# Autodesk Inventor assembly: Pancake_Timing Assy_Star Shaft 2_3 Lanes
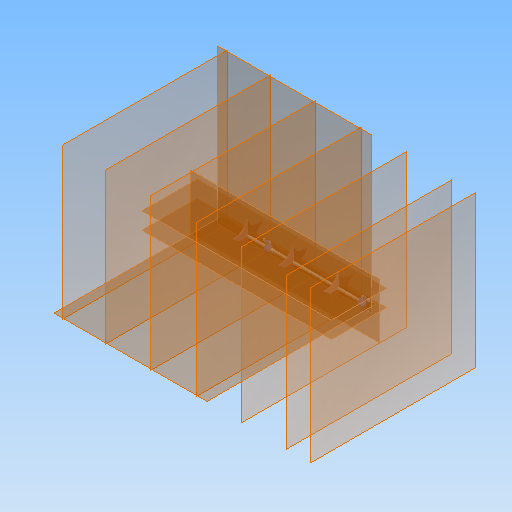
[picture p0: Inventor's stored thumbnail of the model, 512x512]
Saved by Autodesk Inventor 2018.1 (Build 221171000, 171)
## iProperties
Created: 2019-02-11
Part Number: Pancake_Timing Assy_Star Shaft 2_3 Lanes
Document SubType Name: Assembly
Designer: James
Mass: 92.827 g
Surface Area: 261.339 cm^2
Volume: 33.0472 cm^3
Density: 2.80892 g/cm^3
Author: James
## Documents named in this file (7)
- C:\Users\admin\Desktop\Ball-Machine\Pancake Sort\Pancake - 3 Lanes\Pancake_Timing Assy_Star Shaft 2_3 Lanes.iam
- C:\Users\admin\Desktop\Ball-Machine\Pancake Sort\BS 3673 - 6mm External Circlip.ipt
- C:\Users\admin\Desktop\Ball-Machine\Timing Gate\SAFL212 Oval 2 Bolt Flanged Unit.ipt
- C:\Users\admin\Desktop\Ball-Machine\Pancake Sort\Locknut - M3.ipt
- C:\Users\admin\Desktop\Ball-Machine\Pancake Sort\Socket Cap Screw - Standard - (A2) - M3 x 12.ipt
- C:\Users\admin\Desktop\Ball-Machine\Timing Gate\Timing_Star.ipt
- C:\Users\admin\Desktop\Ball-Machine\Pancake Sort\Pancake - 3 Lanes\Pancake_Star Shaft 2_3 Lanes.ipt
## Components (19 placed, 6 different names)
1. Pancake_Star Shaft 2_3 Lanes:1 — Mate:4, Mate:49, Mate:50, Mate:61, Mate:62, Mate:63, Mate:66, Mate:68, Flush:29
2. SAFL212 Oval 2 Bolt Flanged Unit:1 — Mate:61, Flush:24, Angle:4, Mate:65, Mate:79, Mate:80, Mate:81, Mate:82, Mate:83
3. SAFL212 Oval 2 Bolt Flanged Unit:2 — Mate:62, Flush:24, Mate:64, Mate:74, Mate:75, Mate:76, Mate:77, Mate:78, Flush:29
4. BS 3673 - 6mm External Circlip:16 — Mate:65, Mate:66, Flush:25, Mate:68
5. BS 3673 - 6mm External Circlip:17 — Mate:63, Mate:64, Flush:25, Flush:26
6. Locknut - M3:1 — Flush:27, Mate:78
7. Socket Cap Screw - Standard - (A2) - M3 x 12:1 — Mate:74, Mate:77
8. Locknut - M3:2 — Flush:27
9. Socket Cap Screw - Standard - (A2) - M3 x 12:2 — Mate:75, Mate:76
10. Locknut - M3:3 — Flush:28, Mate:83
11. Socket Cap Screw - Standard - (A2) - M3 x 12:3 — Mate:79, Mate:81
12. Locknut - M3:4 — Flush:28
13. Socket Cap Screw - Standard - (A2) - M3 x 12:4 — Mate:80, Mate:82
14. BS 3673 - 6mm External Circlip:11 — Mate:49, Mate:50, Flush:26, Mate:69
15. Timing_Star:1 — Mate:4, Mate:69
16. BS 3673 - 6mm External Circlip:12
17. Timing_Star:2
18. BS 3673 - 6mm External Circlip:13
19. Timing_Star:3
## Component patterns: (3 elements, first: BS 3673 - 6mm External Circlip:11 + Timing_Star:1)
## Relationships (39: Mate 25, Flush 12, Angle 2)
- Mate:4: Pancake_Star Shaft 2_3 Lanes:1 ↔ Timing_Star:1
- [Flush]: Pancake_Star Shaft 2_3 Lanes:1
- Flush:11 (-58 mm)
- Flush:12 (-5 mm)
- Flush:13 (30 mm)
- [Flush]: Pancake_Star Shaft 2_3 Lanes:1
- [Flush]: Pancake_Star Shaft 2_3 Lanes:1
- Mate:49: Pancake_Star Shaft 2_3 Lanes:1 ↔ BS 3673 - 6mm External Circlip:11
- Mate:50: Pancake_Star Shaft 2_3 Lanes:1 ↔ BS 3673 - 6mm External Circlip:11
- [Angle] (0 deg): Pancake_Star Shaft 2_3 Lanes:1 ↔ BS 3673 - 6mm External Circlip:11
- Mate:61: Pancake_Star Shaft 2_3 Lanes:1 ↔ SAFL212 Oval 2 Bolt Flanged Unit:1
- Mate:62: Pancake_Star Shaft 2_3 Lanes:1 ↔ SAFL212 Oval 2 Bolt Flanged Unit:2
- Flush:24: SAFL212 Oval 2 Bolt Flanged Unit:1 ↔ SAFL212 Oval 2 Bolt Flanged Unit:2
- Angle:4 (0 deg): SAFL212 Oval 2 Bolt Flanged Unit:1
- Mate:63: Pancake_Star Shaft 2_3 Lanes:1 ↔ BS 3673 - 6mm External Circlip:17
- Mate:64: SAFL212 Oval 2 Bolt Flanged Unit:2 ↔ BS 3673 - 6mm External Circlip:17
- Mate:65: SAFL212 Oval 2 Bolt Flanged Unit:1 ↔ BS 3673 - 6mm External Circlip:16
- Mate:66: Pancake_Star Shaft 2_3 Lanes:1 ↔ BS 3673 - 6mm External Circlip:16
- Flush:25: BS 3673 - 6mm External Circlip:16 ↔ BS 3673 - 6mm External Circlip:17
- Flush:26: BS 3673 - 6mm External Circlip:17 ↔ BS 3673 - 6mm External Circlip:11
- Mate:69: BS 3673 - 6mm External Circlip:11 ↔ Timing_Star:1
- Mate:68: Pancake_Star Shaft 2_3 Lanes:1 ↔ BS 3673 - 6mm External Circlip:16
- [Mate]: Locknut - M3:1 ↔ Socket Cap Screw - Standard - (A2) - M3 x 12:1
- [Mate]: Locknut - M3:2 ↔ Socket Cap Screw - Standard - (A2) - M3 x 12:2
- [Mate]: Locknut - M3:3 ↔ Socket Cap Screw - Standard - (A2) - M3 x 12:3
- [Mate]: Locknut - M3:4 ↔ Socket Cap Screw - Standard - (A2) - M3 x 12:4
- Mate:74: SAFL212 Oval 2 Bolt Flanged Unit:2 ↔ Socket Cap Screw - Standard - (A2) - M3 x 12:1
- Mate:75: SAFL212 Oval 2 Bolt Flanged Unit:2 ↔ Socket Cap Screw - Standard - (A2) - M3 x 12:2
- Mate:76: SAFL212 Oval 2 Bolt Flanged Unit:2 ↔ Socket Cap Screw - Standard - (A2) - M3 x 12:2
- Mate:77: SAFL212 Oval 2 Bolt Flanged Unit:2 ↔ Socket Cap Screw - Standard - (A2) - M3 x 12:1
- Flush:27: Locknut - M3:1 ↔ Locknut - M3:2
- Mate:78 (3 mm): SAFL212 Oval 2 Bolt Flanged Unit:2 ↔ Locknut - M3:1
- Mate:79: SAFL212 Oval 2 Bolt Flanged Unit:1 ↔ Socket Cap Screw - Standard - (A2) - M3 x 12:3
- Mate:80: SAFL212 Oval 2 Bolt Flanged Unit:1 ↔ Socket Cap Screw - Standard - (A2) - M3 x 12:4
- Mate:81: SAFL212 Oval 2 Bolt Flanged Unit:1 ↔ Socket Cap Screw - Standard - (A2) - M3 x 12:3
- Mate:82: SAFL212 Oval 2 Bolt Flanged Unit:1 ↔ Socket Cap Screw - Standard - (A2) - M3 x 12:4
- Flush:28: Locknut - M3:3 ↔ Locknut - M3:4
- Mate:83 (3 mm): SAFL212 Oval 2 Bolt Flanged Unit:1 ↔ Locknut - M3:3
- Flush:29: Pancake_Star Shaft 2_3 Lanes:1 ↔ SAFL212 Oval 2 Bolt Flanged Unit:2
## Named parameters: d156_d65 = 0 mm, d157_d65 = 0 mm, d158_d65 = 0 mm
